# Autodesk Inventor assembly: boxxing
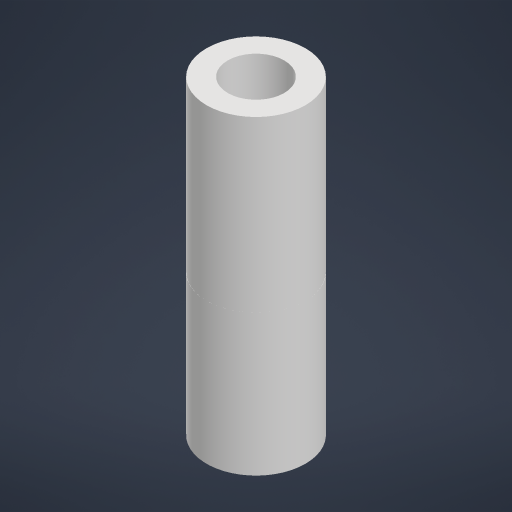
[picture p0: Inventor's stored thumbnail of the model, 512x512]
Saved by Autodesk Inventor 2024 (Build 280153000, 153)
## iProperties
Created: 2024-01-04
Part Number: boxxing
Document SubType Name: Assembly
Designer: macbook
Author: macbook
## Documents named in this file (3)
- \\Mac\Home\Desktop\code\1599V-VRC\Cad\Assembly\boxxing.iam
- \\Mac\Home\Desktop\code\1599V-VRC\Cad\Assembly\10mm spacer.ipt
- \\Mac\Home\Desktop\code\1599V-VRC\Cad\Assembly\12mm spacer.ipt
## Components (2 placed, 2 different names)
1. 10mm spacer:1 — Insert:1
2. 12mm spacer:1 — Insert:1
## Relationships (1: Insert 1)
- Insert:1: 10mm spacer:1 ↔ 12mm spacer:1
